# Autodesk Inventor assembly: 15102898-16-A-0200
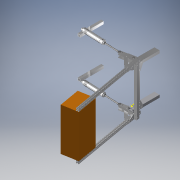
[picture p0: Inventor's stored thumbnail of the model, 180x180]
Saved by Autodesk Inventor 2017 (Build 210142000, 142)
## iProperties
Created: 2016-09-26
Part Number: 15102898-16-A-0200
Document SubType Name: Assembly
Designer: gus
Mass: 4256.38 g
Surface Area: 9011.94 cm^2
Volume: 1308.67 cm^3
Density: 3.25244 g/cm^3
Author: gus
## Documents named in this file (20)
- \\Mac\Home\Desktop\bunnybots 2016\15102898-16-Bunnybot-CAD\Bunnybot-To_be_renamed\15102898-16-A-0000\15102898-16-A-0200\15102898-16-A-0200.iam
- \\Mac\Home\Desktop\bunnybots 2016\15102898-16-Bunnybot-CAD\Bunnybot-To_be_renamed\15102898-16-A-0000\15102898-16-A-0200\15102898-16-P-0201.ipt
- \\Mac\Home\Desktop\bunnybots 2016\15102898-16-Bunnybot-CAD\Bunnybot-To_be_renamed\15102898-16-A-0000\15102898-16-A-0200\Imported Components\217-2732.20121205.ipt
- \\Mac\Home\Desktop\bunnybots 2016\15102898-16-Bunnybot-CAD\Bunnybot-To_be_renamed\15102898-16-A-0000\15102898-16-A-0200\Imported Components\8020-1010.ipt
- \\Mac\Home\Desktop\bunnybots 2016\15102898-16-Bunnybot-CAD\Bunnybot-To_be_renamed\15102898-16-A-0000\15102898-16-A-0200\15102898-16-P-0201_MIR.ipt
- \\Mac\Home\Desktop\bunnybots 2016\15102898-16-Bunnybot-CAD\Bunnybot-To_be_renamed\15102898-16-A-0000\15102898-16-A-0200\Imported Components\217-2732.20121205_MIR.ipt
- \\Mac\Home\Desktop\bunnybots 2016\15102898-16-Bunnybot-CAD\Bunnybot-To_be_renamed\15102898-16-A-0000\15102898-16-A-0200\Imported Components\8020-1010_MIR.ipt
- \\Mac\Home\Desktop\bunnybots 2016\15102898-16-Bunnybot-CAD\Bunnybot-To_be_renamed\15102898-16-A-0000\15102898-16-A-0200\15102898-16-P-0203.ipt
- \\Mac\Home\Desktop\bunnybots 2016\15102898-16-Bunnybot-CAD\Bunnybot-To_be_renamed\15102898-16-A-0000\15102898-16-A-0200\15102898-16-A-0205.ipt
- \\Mac\Home\Desktop\bunnybots 2016\15102898-16-Bunnybot-CAD\Bunnybot-To_be_renamed\15102898-16-A-0000\15102898-16-A-0200\AIS2015\175-DPEE5(F,D-231-1).iam
- \\Mac\Home\Desktop\bunnybots 2016\15102898-16-Bunnybot-CAD\Bunnybot-To_be_renamed\15102898-16-A-0000\15102898-16-A-0200\15102898-16-A-0204.iam
- \\Mac\Home\Desktop\bunnybots 2016\15102898-16-Bunnybot-CAD\Bunnybot-To_be_renamed\15102898-16-A-0000\15102898-16-A-0200\15102898-16-P-0205.ipt
- \\Mac\Home\Desktop\bunnybots 2016\15102898-16-Bunnybot-CAD\Bunnybot-To_be_renamed\15102898-16-A-0000\15102898-16-A-0200\Imported Components\91257A636_HIGH-STRENGTH GRADE 8 STEEL CAP SCREW.ipt
- \\Mac\Home\Desktop\bunnybots 2016\15102898-16-Bunnybot-CAD\Bunnybot-To_be_renamed\15102898-16-A-0000\15102898-16-A-0200\Imported Components\97135A230_GRADE 8 STEEL NYLON-INSERT LOCKNUT.ipt
- \\Mac\Home\Desktop\bunnybots 2016\15102898-16-Bunnybot-CAD\Bunnybot-To_be_renamed\15102898-16-A-0000\15102898-16-A-0200\15102898-16-P-0206.ipt
- \\Mac\Home\Desktop\bunnybots 2016\15102898-16-Bunnybot-CAD\Bunnybot-To_be_renamed\15102898-16-A-0000\15102898-16-A-0200\15102898-16-P-0207.ipt
- \\Mac\Home\Desktop\bunnybots 2016\15102898-16-Bunnybot-CAD\Bunnybot-To_be_renamed\15102898-16-A-0000\15102898-16-A-0200\15102898-16-P-0208.ipt
- \\Mac\Home\Desktop\bunnybots 2016\15102898-16-Bunnybot-CAD\Bunnybot-To_be_renamed\15102898-16-A-0000\15102898-16-A-0200\15102898-16-P-0209.ipt
- \\Mac\Home\Desktop\bunnybots 2016\15102898-16-Bunnybot-CAD\Bunnybot-To_be_renamed\15102898-16-A-0000\15102898-16-A-0200\15102898-16-P-0210.ipt
- \\Mac\Home\Desktop\bunnybots 2016\15102898-16-Bunnybot-CAD\Bunnybot-To_be_renamed\15102898-16-A-0000\15102898-16-A-0200\placeholder for bucket.ipt
## Components (31 placed, 19 different names)
1. 15102898-16-P-0201:1 — Mate:1, Mate:4, Mate:5, Flush:9, Flush:10, Mate:14, Mate:32, Mate:42, Flush:34, Flush:35, Flush:36
2. 217-2732.20121205:1 — Mate:1, Mate:4, Mate:5, Cylindrical:6, Mate:22
3. 8020-1010:1 — Flush:11, Mate:19, Flush:13, Flush:25, Flush:29, Flush:30, Flush:38, Flush:39
4. 15102898-16-P-0201_MIR:1 — Flush:3, Mate:6, Mate:8, Flush:24, Mate:31, Mate:41, Flush:33, Flush:37
5. 217-2732.20121205_MIR:1 — Flush:3, Mate:6, Mate:8, Cylindrical:7, Mate:27
6. 8020-1010_MIR:1 — Flush:19, Mate:24, Mate:25, Flush:26, Mate:40, Flush:32, Mate:46, Flush:50, Mate:49, Mate:50
7. 15102898-16-P-0203:1 — Cylindrical:5, Mate:17, Flush:11, Mate:20, Mate:21, Cylindrical:6, Flush:40, Mate:47
8. 15102898-16-A-0205:1 — Flush:9, Flush:10, Mate:14, Mate:16, Flush:22, Flush:23
9. 175-DPEE5(F,D-231-1):1 [sub-assembly] — Mate:16, Cylindrical:4
10. 15102898-16-A-0204:1 [sub-assembly] — Cylindrical:4, Cylindrical:5, Mate:17
11. 15102898-16-P-0205:1 — Mate:19, Flush:13, Cylindrical:12, Mate:33, Mate:34, Mate:37, Flush:41, Mate:51
12. 15102898-16-P-0205:2 — Flush:21, Mate:24, Mate:26, Mate:27, Flush:42, Flush:50
13. 15102898-16-P-0205:3 — Flush:19, Flush:21, Mate:25, Cylindrical:13, Mate:30, Flush:51, Mate:49
14. 15102898-16-P-0205:4 — Mate:20, Mate:21, Mate:22, Flush:40, Flush:41
15. 15102898-16-P-0203:2 — Cylindrical:7, Mate:26, Cylindrical:9, Mate:29, Flush:42, Flush:51
16. 15102898-16-A-0205:2 — Flush:22, Flush:23, Flush:24
17. 175-DPEE5(F,D-231-1):2 [sub-assembly]
18. 15102898-16-A-0204:2 [sub-assembly] — Cylindrical:9, Mate:29
19. 91257A636_HIGH-STRENGTH GRADE 8 STEEL CAP SCREW:1 — Cylindrical:10, Cylindrical:13, Mate:30
20. 91257A636_HIGH-STRENGTH GRADE 8 STEEL CAP SCREW:2 — Cylindrical:11, Cylindrical:12, Mate:33, Mate:47
21. 97135A230_GRADE 8 STEEL NYLON-INSERT LOCKNUT:1 — Cylindrical:10, Mate:31
22. 97135A230_GRADE 8 STEEL NYLON-INSERT LOCKNUT:2 — Cylindrical:11, Mate:32
23. 15102898-16-P-0206:1 — Flush:25, Mate:34, Mate:35, Flush:27, Flush:28, Mate:36, Mate:38, Flush:31, Mate:39
24. 15102898-16-P-0207:1 — Flush:26, Mate:35, Flush:27, Mate:50
25. 15102898-16-P-0207:2 — Flush:28, Mate:36, Mate:37, Flush:29, Mate:51
26. 15102898-16-P-0208:1 — Flush:30, Mate:38, Flush:31
27. 15102898-16-P-0208:2 — Mate:39, Mate:40, Flush:32
28. 15102898-16-P-0209:1 — Mate:41, Flush:33, Mate:42, Flush:34, Mate:43, Mate:44, Mate:45
29. 15102898-16-P-0210:1 — Flush:35, Flush:36, Mate:43
30. 15102898-16-P-0210:2 — Mate:44, Flush:37, Mate:45
31. placeholder for bucket:1 — Mate:46, Flush:38, Flush:39
## Relationships (79: Mate 39, Flush 30, CylindricalJoint 10)
- Mate:1: 15102898-16-P-0201:1 ↔ 217-2732.20121205:1
- Mate:4: 15102898-16-P-0201:1 ↔ 217-2732.20121205:1
- Mate:5: 15102898-16-P-0201:1 ↔ 217-2732.20121205:1
- Flush:3: 15102898-16-P-0201_MIR:1 ↔ 217-2732.20121205_MIR:1
- Mate:6: 15102898-16-P-0201_MIR:1 ↔ 217-2732.20121205_MIR:1
- Mate:8: 15102898-16-P-0201_MIR:1 ↔ 217-2732.20121205_MIR:1
- Flush:9: 15102898-16-P-0201:1 ↔ 15102898-16-A-0205:1
- Flush:10: 15102898-16-P-0201:1 ↔ 15102898-16-A-0205:1
- Mate:14 (467.995 mm): 15102898-16-P-0201:1 ↔ 15102898-16-A-0205:1
- Mate:16: 15102898-16-A-0205:1 ↔ 175-DPEE5(F,D-231-1):1
- Cylindrical:4: 175-DPEE5(F,D-231-1):1 ↔ 15102898-16-A-0204:1
- Cylindrical:5: 15102898-16-P-0203:1 ↔ 15102898-16-A-0204:1
- Mate:17: 15102898-16-P-0203:1 ↔ 15102898-16-A-0204:1
- Flush:11: 8020-1010:1 ↔ 15102898-16-P-0203:1
- Mate:19: 8020-1010:1 ↔ 15102898-16-P-0205:1
- Flush:13: 8020-1010:1 ↔ 15102898-16-P-0205:1
- Mate:20: 15102898-16-P-0203:1 ↔ 15102898-16-P-0205:4
- Mate:21: 15102898-16-P-0203:1 ↔ 15102898-16-P-0205:4
- Cylindrical:6: 217-2732.20121205:1 ↔ 15102898-16-P-0203:1
- Mate:22 (3.175 mm): 217-2732.20121205:1 ↔ 15102898-16-P-0205:4
- Flush:19: 8020-1010_MIR:1 ↔ 15102898-16-P-0205:3
- Flush:21: 15102898-16-P-0205:2 ↔ 15102898-16-P-0205:3
- Mate:24: 8020-1010_MIR:1 ↔ 15102898-16-P-0205:2
- Mate:25: 8020-1010_MIR:1 ↔ 15102898-16-P-0205:3
- Cylindrical:7: 217-2732.20121205_MIR:1 ↔ 15102898-16-P-0203:2
- Mate:26: 15102898-16-P-0205:2 ↔ 15102898-16-P-0203:2
- Mate:27 (3.175 mm): 217-2732.20121205_MIR:1 ↔ 15102898-16-P-0205:2
- [Mate]: 15102898-16-A-0205:2 ↔ 175-DPEE5(F,D-231-1):2
- [CylindricalJoint]: 175-DPEE5(F,D-231-1):2 ↔ 15102898-16-A-0204:2
- Flush:22: 15102898-16-A-0205:1 ↔ 15102898-16-A-0205:2
- Flush:23: 15102898-16-A-0205:1 ↔ 15102898-16-A-0205:2
- Flush:24: 15102898-16-P-0201_MIR:1 ↔ 15102898-16-A-0205:2
- Cylindrical:9: 15102898-16-P-0203:2 ↔ 15102898-16-A-0204:2
- Mate:29: 15102898-16-P-0203:2 ↔ 15102898-16-A-0204:2
- Cylindrical:10: 91257A636_HIGH-STRENGTH GRADE 8 STEEL CAP SCREW:1 ↔ 97135A230_GRADE 8 STEEL NYLON-INSERT LOCKNUT:1
- Cylindrical:11: 91257A636_HIGH-STRENGTH GRADE 8 STEEL CAP SCREW:2 ↔ 97135A230_GRADE 8 STEEL NYLON-INSERT LOCKNUT:2
- Cylindrical:12: 15102898-16-P-0205:1 ↔ 91257A636_HIGH-STRENGTH GRADE 8 STEEL CAP SCREW:2
- Cylindrical:13: 15102898-16-P-0205:3 ↔ 91257A636_HIGH-STRENGTH GRADE 8 STEEL CAP SCREW:1
- Mate:30: 15102898-16-P-0205:3 ↔ 91257A636_HIGH-STRENGTH GRADE 8 STEEL CAP SCREW:1
- Mate:31: 15102898-16-P-0201_MIR:1 ↔ 97135A230_GRADE 8 STEEL NYLON-INSERT LOCKNUT:1
- Mate:32: 15102898-16-P-0201:1 ↔ 97135A230_GRADE 8 STEEL NYLON-INSERT LOCKNUT:2
- Mate:33: 15102898-16-P-0205:1 ↔ 91257A636_HIGH-STRENGTH GRADE 8 STEEL CAP SCREW:2
- Flush:25: 8020-1010:1 ↔ 15102898-16-P-0206:1
- Mate:34: 15102898-16-P-0205:1 ↔ 15102898-16-P-0206:1
- Flush:26: 8020-1010_MIR:1 ↔ 15102898-16-P-0207:1
- Mate:35: 15102898-16-P-0206:1 ↔ 15102898-16-P-0207:1
- Flush:27: 15102898-16-P-0206:1 ↔ 15102898-16-P-0207:1
- Flush:28: 15102898-16-P-0206:1 ↔ 15102898-16-P-0207:2
- Mate:36: 15102898-16-P-0206:1 ↔ 15102898-16-P-0207:2
- Mate:37: 15102898-16-P-0205:1 ↔ 15102898-16-P-0207:2
- Flush:29: 8020-1010:1 ↔ 15102898-16-P-0207:2
- Flush:30: 8020-1010:1 ↔ 15102898-16-P-0208:1
- Mate:38: 15102898-16-P-0206:1 ↔ 15102898-16-P-0208:1
- Flush:31: 15102898-16-P-0206:1 ↔ 15102898-16-P-0208:1
- Mate:39: 15102898-16-P-0206:1 ↔ 15102898-16-P-0208:2
- Mate:40: 8020-1010_MIR:1 ↔ 15102898-16-P-0208:2
- Flush:32: 8020-1010_MIR:1 ↔ 15102898-16-P-0208:2
- Mate:41: 15102898-16-P-0201_MIR:1 ↔ 15102898-16-P-0209:1
- Flush:33: 15102898-16-P-0201_MIR:1 ↔ 15102898-16-P-0209:1
- Mate:42: 15102898-16-P-0201:1 ↔ 15102898-16-P-0209:1
- Flush:34 (38.1 mm): 15102898-16-P-0201:1 ↔ 15102898-16-P-0209:1
- Flush:35: 15102898-16-P-0201:1 ↔ 15102898-16-P-0210:1
- Flush:36: 15102898-16-P-0201:1 ↔ 15102898-16-P-0210:1
- Mate:43: 15102898-16-P-0209:1 ↔ 15102898-16-P-0210:1
- Mate:44: 15102898-16-P-0209:1 ↔ 15102898-16-P-0210:2
- Flush:37: 15102898-16-P-0201_MIR:1 ↔ 15102898-16-P-0210:2
- Mate:45: 15102898-16-P-0209:1 ↔ 15102898-16-P-0210:2
- Mate:46: 8020-1010_MIR:1 ↔ placeholder for bucket:1
- Flush:38: 8020-1010:1 ↔ placeholder for bucket:1
- Flush:39: 8020-1010:1 ↔ placeholder for bucket:1
- Flush:40: 15102898-16-P-0203:1 ↔ 15102898-16-P-0205:4
- Mate:47: 15102898-16-P-0203:1 ↔ 91257A636_HIGH-STRENGTH GRADE 8 STEEL CAP SCREW:2
- Flush:41: 15102898-16-P-0205:1 ↔ 15102898-16-P-0205:4
- Flush:42: 15102898-16-P-0205:2 ↔ 15102898-16-P-0203:2
- Flush:50: 8020-1010_MIR:1 ↔ 15102898-16-P-0205:2
- Flush:51: 15102898-16-P-0205:3 ↔ 15102898-16-P-0203:2
- Mate:49: 8020-1010_MIR:1 ↔ 15102898-16-P-0205:3
- Mate:50: 8020-1010_MIR:1 ↔ 15102898-16-P-0207:1
- Mate:51: 15102898-16-P-0205:1 ↔ 15102898-16-P-0207:2
## Named parameters: d114_d59 = 0 mm, d115_d66 = 0 deg, d116_d67 = 101.6 mm, d117_d68 = 101.55448 mm, d118_d69 = -25.4 mm
